# Autodesk Inventor assembly: GI - 200
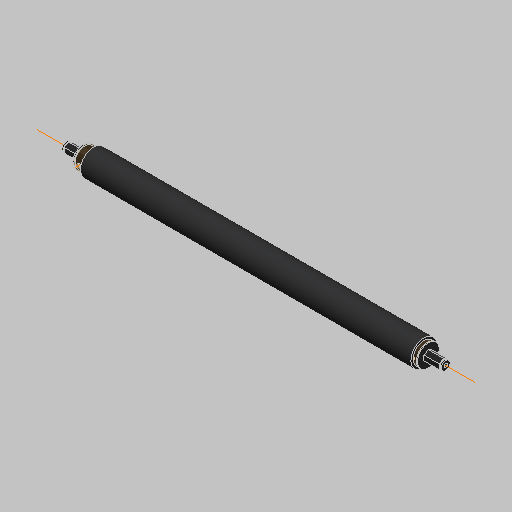
[picture p0: Inventor's stored thumbnail of the model, 512x512]
Saved by Autodesk Inventor 2023.5 (Build 275446000, 446)
## iProperties
Created: 2025-01-18
Part Number: GI - 200
Document SubType Name: Assembly
Designer: mavericks
Mass: 311.701 g
Surface Area: 2121.29 cm^2
Volume: 267.774 cm^3
Density: 1.16404 g/cm^3
Author: mavericks
## Documents named in this file (4)
- C:\Users\slick\OneDrive\Desktop\2025-ReefScape---CAD\ground intake\GI - 200.iam
- C:\Users\slick\OneDrive\Desktop\2025-ReefScape---CAD\ground intake\GI1\GI - 003.ipt
- C:\Users\slick\OneDrive\Desktop\2025-ReefScape---CAD\ground intake\GI1\GI - 004.ipt
- C:\Users\slick\OneDrive\Desktop\2025-ReefScape---CAD\COMMON PARTS\WCP\WCP-0102.ipt
## Components (4 placed, 3 different names)
1. GI - 003:1 — Insert:1, Insert:2, Mate:1, Mate:3, Mate:4, Mate:5, Mate:6
2. WCP-0102:1 — Insert:1, Mate:4, Mate:5
3. WCP-0102:2 — Insert:2, Mate:2, Mate:3, Mate:6
4. GI - 004:1 — Mate:1, Mate:2
## Relationships (8: Mate 6, Insert 2)
- Insert:1: GI - 003:1 ↔ WCP-0102:1
- Insert:2: GI - 003:1 ↔ WCP-0102:2
- Mate:1: GI - 003:1 ↔ GI - 004:1
- Mate:2: WCP-0102:2 ↔ GI - 004:1
- Mate:3: GI - 003:1 ↔ WCP-0102:2
- Mate:4: GI - 003:1 ↔ WCP-0102:1
- Mate:5: GI - 003:1 ↔ WCP-0102:1
- Mate:6: GI - 003:1 ↔ WCP-0102:2
